# Autodesk Inventor assembly: gyroPhone03
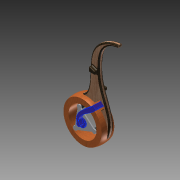
[picture p0: Inventor's stored thumbnail of the model, 180x180]
Saved by Autodesk Inventor 2013 (Build 170138000, 138)
## iProperties
Created: 2013-01-09
Part Number: gyroPhone03
Document SubType Name: Assembly
Designer: Nano
Author: Nano
## Documents named in this file (6)
- C:\Users\Nano\Documents\InventorByron\InventorMasterProject\gyroPhone01\gyroPhone03.iam
- C:\Users\Nano\Documents\InventorByron\InventorMasterProject\gyroPhone01\bodyMainAirPipe.ipt
- C:\Users\Nano\Documents\InventorByron\InventorMasterProject\gyroPhone01\fork.ipt
- C:\Users\Nano\Documents\InventorByron\InventorMasterProject\gyroPhone01\motorPlate.ipt
- C:\Users\Nano\Documents\InventorByron\InventorMasterProject\gyroPhone01\motorAssembly01.iam
- C:\Users\Nano\Documents\InventorByron\InventorMasterProject\gyroPhone01\bigWheel.ipt
## Components (7 placed, 5 different names)
1. bodyMainAirPipe:1 — Mate:1, Mate:2, parallelWheelInBody
2. fork:1 — Mate:1, Mate:2, Mate:3, Mate:4, Angle:1
3. motorPlate:1 — Mate:3, Mate:4, Angle:1, Mate:5, Mate:6, Mate:7, Mate:8, Mate:9, Mate:10, Mate:11, parallelWheelInBody
4. motorAssembly01:1 [sub-assembly] — Mate:5, Mate:6, Flush:1
5. motorAssembly01:2 [sub-assembly] — Mate:7, Mate:8
6. motorAssembly01:3 [sub-assembly] — Mate:9, Mate:10
7. bigWheel:1 — Mate:11, Flush:1
## Relationships (14: Mate 11, Angle 2, Flush 1)
- Mate:1: bodyMainAirPipe:1 ↔ fork:1
- Mate:2: bodyMainAirPipe:1 ↔ fork:1
- Mate:3: fork:1 ↔ motorPlate:1
- Mate:4: fork:1 ↔ motorPlate:1
- Angle:1 (0 deg): fork:1 ↔ motorPlate:1
- Mate:5: motorPlate:1 ↔ motorAssembly01:1
- Mate:6: motorPlate:1 ↔ motorAssembly01:1
- Mate:7: motorPlate:1 ↔ motorAssembly01:2
- Mate:8: motorPlate:1 ↔ motorAssembly01:2
- Mate:9: motorPlate:1 ↔ motorAssembly01:3
- Mate:10: motorPlate:1 ↔ motorAssembly01:3
- Mate:11: motorPlate:1 ↔ bigWheel:1
- Flush:1 (31.75 mm): motorAssembly01:1 ↔ bigWheel:1
- parallelWheelInBody [Angle] (0 deg): bodyMainAirPipe:1 ↔ motorPlate:1
